# Autodesk Inventor assembly: Tapicerka_oparcia
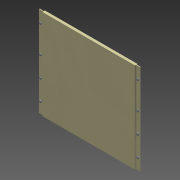
[picture p0: Inventor's stored thumbnail of the model, 180x180]
Saved by Autodesk Inventor 2014 SP2 (Build 180246200, 246)
## iProperties
Created: 2015-12-07
Part Number: Tapicerka_oparcia
Document SubType Name: Assembly
Designer: graaapsik
Author: graaapsik
## Documents named in this file (6)
- G:\Dokumenty\♥ MECHANIKA\2 semestr\ZSW CAD CAM CAE\Projekt\Model\Tapicerka_oparcia.iam
- G:\Dokumenty\♥ MECHANIKA\2 semestr\ZSW CAD CAM CAE\Projekt\Model\Listwa_oparcia.ipt
- G:\Dokumenty\♥ MECHANIKA\2 semestr\ZSW CAD CAM CAE\Projekt\Model\Pianka_oparcia.ipt
- G:\Dokumenty\♥ MECHANIKA\2 semestr\ZSW CAD CAM CAE\Projekt\Model\Tapicerka_oparcia.ipt
- G:\Dokumenty\♥ MECHANIKA\2 semestr\ZSW CAD CAM CAE\Projekt\Model\ISO 7092 - ST 6 - 140 HV.ipt
- G:\Dokumenty\♥ MECHANIKA\2 semestr\ZSW CAD CAM CAE\Projekt\Model\ISO 7380 - M6 x 10.ipt
## Components (20 placed, 5 different names)
1. Tapicerka_oparcia:1 — Zestawiający:1, Zestawiający:2, Zestawiający:3, Zestawiający:4, Zestawiający:5, Zestawiający:6, Zestawiający:7, Wstaw:1, Wstaw:2, Wstaw:3, Wstaw:4, Wstaw:5, Wstaw:6, Wstaw:7, Wstaw:8
2. Pianka_oparcia:1 — Zestawiający:1, Zestawiający:2, Zestawiający:3
3. Listwa_oparcia:1 — Równoległy:1, Równoległy:2, Zestawiający:7
4. Listwa_oparcia:2 — Równoległy:1, Równoległy:2, Zestawiający:4, Zestawiający:5, Zestawiający:6
5. ISO 7092 ST 6 - 140 HV:1 — Wstaw:1, Wstaw:9
6. ISO 7092 ST 6 - 140 HV:2 — Wstaw:2, Wstaw:14
7. ISO 7092 ST 6 - 140 HV:3 — Wstaw:3, Wstaw:13
8. ISO 7092 ST 6 - 140 HV:4 — Wstaw:4, Wstaw:10
9. ISO 7092 ST 6 - 140 HV:5 — Wstaw:5, Wstaw:12
10. ISO 7092 ST 6 - 140 HV:6 — Wstaw:6, Wstaw:11
11. ISO 7092 ST 6 - 140 HV:7 — Wstaw:7, Zestawiający:8, Zestawiający:9
12. ISO 7092 ST 6 - 140 HV:8 — Wstaw:8, Wstaw:15
13. ISO 7380 M6 x 10:1 — Wstaw:9
14. ISO 7380 M6 x 10:2 — Wstaw:10
15. ISO 7380 M6 x 10:3 — Wstaw:11
16. ISO 7380 M6 x 10:4 — Wstaw:12
17. ISO 7380 M6 x 10:5 — Wstaw:13
18. ISO 7380 M6 x 10:6 — Zestawiający:8, Zestawiający:9
19. ISO 7380 M6 x 10:7 — Wstaw:14
20. ISO 7380 M6 x 10:8 — Wstaw:15
## Relationships (26: Insert 15, Mate 9, Flush 2)
- Zestawiający:1 [Mate] (0.25 mm): Tapicerka_oparcia:1 ↔ Pianka_oparcia:1
- Zestawiający:2 [Mate] (4 mm): Tapicerka_oparcia:1 ↔ Pianka_oparcia:1
- Zestawiający:3 [Mate] (0.25 mm): Tapicerka_oparcia:1 ↔ Pianka_oparcia:1
- Równoległy:1 [Flush]: Listwa_oparcia:1 ↔ Listwa_oparcia:2
- Równoległy:2 [Flush]: Listwa_oparcia:1 ↔ Listwa_oparcia:2
- Zestawiający:4 [Mate]: Tapicerka_oparcia:1 ↔ Listwa_oparcia:2
- Zestawiający:5 [Mate]: Tapicerka_oparcia:1 ↔ Listwa_oparcia:2
- Zestawiający:6 [Mate] (0.25 mm): Tapicerka_oparcia:1 ↔ Listwa_oparcia:2
- Zestawiający:7 [Mate]: Tapicerka_oparcia:1 ↔ Listwa_oparcia:1
- Wstaw:1 [Insert]: Tapicerka_oparcia:1 ↔ ISO 7092 ST 6 - 140 HV:1
- Wstaw:2 [Insert]: Tapicerka_oparcia:1 ↔ ISO 7092 ST 6 - 140 HV:2
- Wstaw:3 [Insert]: Tapicerka_oparcia:1 ↔ ISO 7092 ST 6 - 140 HV:3
- Wstaw:4 [Insert]: Tapicerka_oparcia:1 ↔ ISO 7092 ST 6 - 140 HV:4
- Wstaw:5 [Insert]: Tapicerka_oparcia:1 ↔ ISO 7092 ST 6 - 140 HV:5
- Wstaw:6 [Insert]: Tapicerka_oparcia:1 ↔ ISO 7092 ST 6 - 140 HV:6
- Wstaw:7 [Insert]: Tapicerka_oparcia:1 ↔ ISO 7092 ST 6 - 140 HV:7
- Wstaw:8 [Insert]: Tapicerka_oparcia:1 ↔ ISO 7092 ST 6 - 140 HV:8
- Wstaw:9 [Insert]: ISO 7092 ST 6 - 140 HV:1 ↔ ISO 7380 M6 x 10:1
- Wstaw:10 [Insert]: ISO 7092 ST 6 - 140 HV:4 ↔ ISO 7380 M6 x 10:2
- Wstaw:11 [Insert]: ISO 7092 ST 6 - 140 HV:6 ↔ ISO 7380 M6 x 10:3
- Wstaw:12 [Insert]: ISO 7092 ST 6 - 140 HV:5 ↔ ISO 7380 M6 x 10:4
- Wstaw:13 [Insert]: ISO 7092 ST 6 - 140 HV:3 ↔ ISO 7380 M6 x 10:5
- Zestawiający:8 [Mate]: ISO 7092 ST 6 - 140 HV:7 ↔ ISO 7380 M6 x 10:6
- Zestawiający:9 [Mate]: ISO 7092 ST 6 - 140 HV:7 ↔ ISO 7380 M6 x 10:6
- Wstaw:14 [Insert]: ISO 7092 ST 6 - 140 HV:2 ↔ ISO 7380 M6 x 10:7
- Wstaw:15 [Insert]: ISO 7092 ST 6 - 140 HV:8 ↔ ISO 7380 M6 x 10:8
